# Autodesk Inventor assembly: Lacznik zaokraglony sruby
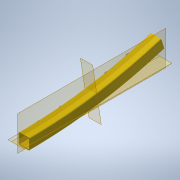
[picture p0: Inventor's stored thumbnail of the model, 180x180]
Saved by Autodesk Inventor 2021 (Build 250183000, 183)
## iProperties
Created: 2024-04-18
Part Number: Lacznik zaokraglony sruby
Document SubType Name: Assembly
Designer: Michal
Author: Michal
## Documents named in this file (3)
- C:\Users\Michal\Documents\GitHub\PNW_PhotoBoothFrame_3D\Lacznik zaokraglony sruby.iam
- C:\Users\Michal\Documents\GitHub\PNW_PhotoBoothFrame_3D\M8x15.ipt
- C:\Users\Michal\Documents\GitHub\PNW_PhotoBoothFrame_3D\Lacznik zaokraglony.ipt
## Components (5 placed, 2 different names)
1. Lacznik zaokraglony:1 — Mate:6, Mate:7, Mate:8, Mate:9, Mate:10
2. M8x15:1 — Flush:1, Flush:2, Flush:3, Mate:10
3. M8x15:2 — Flush:1, Mate:9
4. M8x15:3 — Flush:2, Mate:8
5. M8x15:4 — Flush:3, Mate:6, Mate:7
## Relationships (8: Mate 5, Flush 3)
- Flush:1: M8x15:1 ↔ M8x15:2
- Flush:2: M8x15:1 ↔ M8x15:3
- Flush:3: M8x15:1 ↔ M8x15:4
- Mate:6 (3 mm): Lacznik zaokraglony:1 ↔ M8x15:4
- Mate:7: Lacznik zaokraglony:1 ↔ M8x15:4
- Mate:8: Lacznik zaokraglony:1 ↔ M8x15:3
- Mate:9: Lacznik zaokraglony:1 ↔ M8x15:2
- Mate:10: Lacznik zaokraglony:1 ↔ M8x15:1
